# Autodesk Inventor assembly: PrismMountAdapter
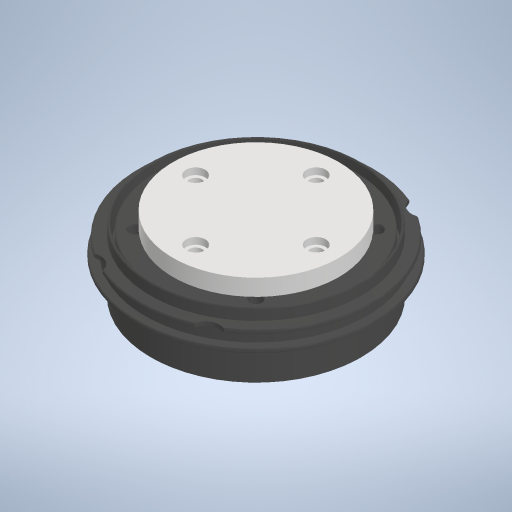
[picture p0: Inventor's stored thumbnail of the model, 512x512]
Saved by Autodesk Inventor 2023 (Build 270158000, 158)
## iProperties
Created: 2024-01-10
Part Number: PrismMountAdapter
Document SubType Name: Assembly
Designer: kerlin
Author: kerlin
## Documents named in this file (3)
- C:\Users\kerlin\Documents\KerlinLab\KTN\Multipass\MechanicalDrawing\PrismMountAdapter.iam
- C:\Users\kerlin\Documents\KerlinLab\KTN\Multipass\MechanicalDrawing\LB4C-Solidworks.ipt
- C:\Users\kerlin\Documents\KerlinLab\KTN\Multipass\MechanicalDrawing\PrismCageAdapter.ipt
## Components (2 placed, 2 different names)
1. LB4C-Solidworks:1 — Mate:1, Mate:2
2. PrismCageAdapter:1 — Mate:1, Mate:2
## Relationships (2: Mate 2)
- Mate:1: LB4C-Solidworks:1 ↔ PrismCageAdapter:1
- Mate:2: LB4C-Solidworks:1 ↔ PrismCageAdapter:1
